# Autodesk Inventor assembly: Fully Integrated CAD System
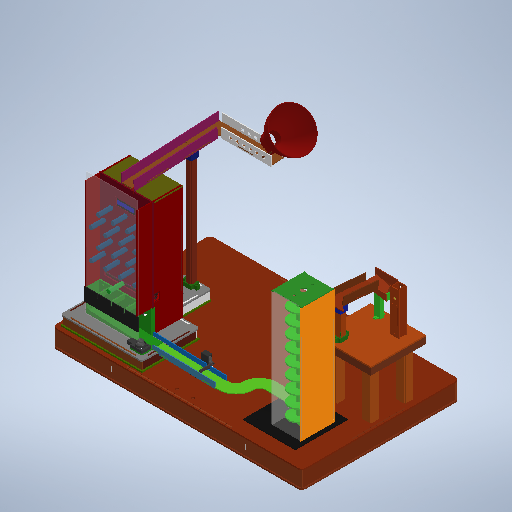
[picture p0: Inventor's stored thumbnail of the model, 512x512]
Saved by Autodesk Inventor 2025.4 (Build 294407000, 407)
## iProperties
Created: 2026-04-11
Part Number: Fully Integrated CAD System
Document SubType Name: Assembly
Designer: lenovo
Author: lenovo
## Documents named in this file (16)
- F:\ASU Engineering\Year.2 ( 25-26 )\Spring\Basics Of Mechatronics\Project\Mechanisms\Fully Integrated CAD System\Fully Integrated CAD System.iam
- F:\ASU Engineering\Year.2 ( 25-26 )\Spring\Basics Of Mechatronics\Project\Mechanisms\Fully Integrated CAD System\Table.ipt
- F:\ASU Engineering\Year.2 ( 25-26 )\Spring\Basics Of Mechatronics\Project\Mechanisms\Sorting Mechanism\Sorting Mechanism Assembly.iam
- F:\ASU Engineering\Year.2 ( 25-26 )\Spring\Basics Of Mechatronics\Project\Mechanisms\Shooting Mechanism\Shooting Assembly FV.iam
- F:\ASU Engineering\Year.2 ( 25-26 )\Spring\Basics Of Mechatronics\Project\Mechanisms\Fully Integrated CAD System\Table-Base Fixation ( Power Port ).ipt
- F:\ASU Engineering\Year.2 ( 25-26 )\Spring\Basics Of Mechatronics\Project\Mechanisms\Fully Integrated CAD System\Table-Base Fixation.ipt
- F:\ASU Engineering\Year.2 ( 25-26 )\Spring\Basics Of Mechatronics\Project\Mechanisms\Fully Integrated CAD System\Table-Base Fixation 2nd.ipt
- F:\ASU Engineering\Year.2 ( 25-26 )\Spring\Basics Of Mechatronics\Project\Mechanisms\Fully Integrated CAD System\Table-Base Supporter 1st.ipt
- F:\ASU Engineering\Year.2 ( 25-26 )\Spring\Basics Of Mechatronics\Project\Mechanisms\Fully Integrated CAD System\Base Full Game.ipt
- F:\ASU Engineering\Year.2 ( 25-26 )\Spring\Basics Of Mechatronics\Project\Mechanisms\Lifting Mechanism\Assembly2.iam
- F:\ASU Engineering\Year.2 ( 25-26 )\Spring\Basics Of Mechatronics\Project\Mechanisms\Fully Integrated CAD System\Starting Path.ipt
- F:\ASU Engineering\Year.2 ( 25-26 )\Spring\Basics Of Mechatronics\Project\Mechanisms\Fully Integrated CAD System\Starting Path Wall.ipt
- F:\ASU Engineering\Year.2 ( 25-26 )\Spring\Basics Of Mechatronics\Project\Mechanisms\Fully Integrated CAD System\Starting Path Wall ( Servo ).ipt
- F:\ASU Engineering\Year.2 ( 25-26 )\Spring\Basics Of Mechatronics\Project\Mechanisms\Fully Integrated CAD System\Servo Housing.ipt
- F:\ASU Engineering\Year.2 ( 25-26 )\Spring\Basics Of Mechatronics\Project\Mechanisms\Fully Integrated CAD System\MS18 MIZUEI SERVO 9G\MS18 MIZUEI SERVO 9G\MS18 MIZUEI SERVO 9G.ipt
- F:\ASU Engineering\Year.2 ( 25-26 )\Spring\Basics Of Mechatronics\Project\Mechanisms\Fully Integrated CAD System\Servo Arm.ipt
## Components (17 placed, 15 different names)
1. Table:1 — Mate:1, Flush:1, Flush:2, Mate:2, Mate:3, Mate:4, Mate:5, Mate:6, Mate:7, Mate:8, Mate:9, Mate:10, Mate:11, Mate:12, Mate:13, Mate:14, Mate:15, Mate:16, Mate:31, Mate:32, Mate:33, Mate:34, Mate:45, Mate:46, Mate:47
2. Sorting Mechanism Assembly:1 [sub-assembly] — Mate:1, Flush:1, Flush:2, Mate:30, Flush:3
3. Shooting Assembly FV:1 [sub-assembly] — Mate:2, Mate:3, Mate:4
4. Table-Base Fixation ( Power Port ):1 — Mate:5, Mate:6, Mate:7
5. Table-Base Fixation:1 — Mate:8, Mate:9, Mate:10
6. Table-Base Fixation 2nd:1 — Mate:11, Mate:12, Mate:13
7. Table-Base Fixation 2nd:3 — Mate:14, Mate:15, Mate:16, Mate:17, Mate:18, Mate:19, Mate:20, Mate:21, Mate:22, Mate:23, Mate:24, Mate:25
8. Table-Base Supporter 1st:1 — Mate:17, Mate:18, Mate:19
9. Table-Base Supporter 1st:2 — Mate:20, Mate:21, Mate:22
10. Base Full Game:1 — Mate:23, Mate:24, Mate:25
11. Assembly2:1 [sub-assembly] — Mate:31, Mate:32, Mate:33, Mate:34
12. Starting Path:1 — Mate:30, Flush:3, Mate:35, Mate:36, Mate:37, Mate:38, Mate:39, Mate:40, Mate:41, Mate:42, Mate:44
13. Starting Path Wall:1 — Mate:35, Mate:36, Mate:37
14. Starting Path Wall ( Servo ):1 — Mate:38, Mate:39, Mate:40
15. Servo Housing:1 — Mate:41, Mate:42, Mate:44, Mate:45, Mate:46, Mate:47, Mate:48, Mate:49, Mate:50
16. MS18 MIZUEI SERVO 9G:1 — Mate:48, Mate:49, Mate:50, Mate:51, Mate:52
17. Servo Arm:1 — Mate:51, Mate:52
## Relationships (50: Mate 47, Flush 3)
- Mate:1: Table:1 ↔ Sorting Mechanism Assembly:1
- Flush:1 (15 mm): Table:1 ↔ Sorting Mechanism Assembly:1
- Flush:2 (15 mm): Table:1 ↔ Sorting Mechanism Assembly:1
- Mate:2: Table:1 ↔ Shooting Assembly FV:1
- Mate:3: Table:1 ↔ Shooting Assembly FV:1
- Mate:4: Table:1 ↔ Shooting Assembly FV:1
- Mate:5: Table:1 ↔ Table-Base Fixation ( Power Port ):1
- Mate:6: Table:1 ↔ Table-Base Fixation ( Power Port ):1
- Mate:7: Table:1 ↔ Table-Base Fixation ( Power Port ):1
- Mate:8: Table:1 ↔ Table-Base Fixation:1
- Mate:9: Table:1 ↔ Table-Base Fixation:1
- Mate:10: Table:1 ↔ Table-Base Fixation:1
- Mate:11: Table:1 ↔ Table-Base Fixation 2nd:1
- Mate:12: Table:1 ↔ Table-Base Fixation 2nd:1
- Mate:13: Table:1 ↔ Table-Base Fixation 2nd:1
- Mate:14: Table:1 ↔ Table-Base Fixation 2nd:3
- Mate:15: Table:1 ↔ Table-Base Fixation 2nd:3
- Mate:16: Table:1 ↔ Table-Base Fixation 2nd:3
- Mate:17: Table-Base Fixation 2nd:3 ↔ Table-Base Supporter 1st:1
- Mate:18: Table-Base Fixation 2nd:3 ↔ Table-Base Supporter 1st:1
- Mate:19: Table-Base Fixation 2nd:3 ↔ Table-Base Supporter 1st:1
- Mate:20: Table-Base Fixation 2nd:3 ↔ Table-Base Supporter 1st:2
- Mate:21: Table-Base Fixation 2nd:3 ↔ Table-Base Supporter 1st:2
- Mate:22: Table-Base Fixation 2nd:3 ↔ Table-Base Supporter 1st:2
- Mate:23: Table-Base Fixation 2nd:3 ↔ Base Full Game:1
- Mate:24: Table-Base Fixation 2nd:3 ↔ Base Full Game:1
- Mate:25: Table-Base Fixation 2nd:3 ↔ Base Full Game:1
- Mate:30: Sorting Mechanism Assembly:1 ↔ Starting Path:1
- Flush:3: Sorting Mechanism Assembly:1 ↔ Starting Path:1
- Mate:31: Table:1 ↔ Assembly2:1
- Mate:32: Table:1 ↔ Assembly2:1
- Mate:33: Table:1 ↔ Assembly2:1
- Mate:34: Table:1 ↔ Assembly2:1
- Mate:35: Starting Path:1 ↔ Starting Path Wall:1
- Mate:36: Starting Path:1 ↔ Starting Path Wall:1
- Mate:37: Starting Path:1 ↔ Starting Path Wall:1
- Mate:38: Starting Path:1 ↔ Starting Path Wall ( Servo ):1
- Mate:39: Starting Path:1 ↔ Starting Path Wall ( Servo ):1
- Mate:40: Starting Path:1 ↔ Starting Path Wall ( Servo ):1
- Mate:41: Starting Path:1 ↔ Servo Housing:1
- Mate:42: Starting Path:1 ↔ Servo Housing:1
- Mate:44: Starting Path:1 ↔ Servo Housing:1
- Mate:45: Table:1 ↔ Servo Housing:1
- Mate:46: Table:1 ↔ Servo Housing:1
- Mate:47: Table:1 ↔ Servo Housing:1
- Mate:48: Servo Housing:1 ↔ MS18 MIZUEI SERVO 9G:1
- Mate:49: Servo Housing:1 ↔ MS18 MIZUEI SERVO 9G:1
- Mate:50: Servo Housing:1 ↔ MS18 MIZUEI SERVO 9G:1
- Mate:51: MS18 MIZUEI SERVO 9G:1 ↔ Servo Arm:1
- Mate:52: MS18 MIZUEI SERVO 9G:1 ↔ Servo Arm:1
